# Autodesk Inventor assembly: Baugruppe1
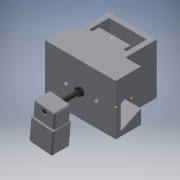
[picture p0: Inventor's stored thumbnail of the model, 180x180]
Saved by Autodesk Inventor 2017 (Build 210142000, 142)
## iProperties
Part Number: Baugruppe1
Material: Generisch
Document SubType Name: Assembly
Designer: Skenderbeg
Author: Skenderbeg
## Documents named in this file (7)
- C:\Users\Skenderbeg\Desktop\Seminar Abschluss\LaserHalterung\Baugruppe1.iam
- C:\Users\Skenderbeg\Desktop\Seminar 2018\21052018 Stick\Freiburg seminar\Schienenaufsatz mitKeil.ipt
- C:\Users\Skenderbeg\Desktop\Seminar 2018\21052018 Stick\Freiburg seminar\Schwalbenschwanz Gegenstück für Cam.ipt
- C:\Users\Skenderbeg\Desktop\Seminar 2018\21052018 Stick\Halterung Laser neu Teil2.ipt
- C:\Users\Skenderbeg\Desktop\Seminar 2018\21052018 Stick\Halterung Neu.ipt
- C:\Users\Skenderbeg\Documents\Inventor\Content Center Files\R2017\de-DE\ISO 7046-1 Z(1)\ISO 7046-1 - M4 x 40 - 4.8 - Z - ISO.ipt
- C:\Users\Skenderbeg\Documents\Inventor\Content Center Files\R2017\de-DE\ISO 4036(2)\ISO 4036 - M4(2).ipt
## Components (6 placed, 6 different names)
1. Schienenaufsatz mitKeil:1 — Verschiebbar:1
2. Schwalbenschwanz Gegenstück für Cam:1 — Verschiebbar:1, Einfügen:1, Einfügen:3
3. Halterung Laser neu Teil2:1 — Starr:1
4. Halterung Neu:1 — Starr:1, Einfügen:2
5. ISO 7046-1 Z M4 x 40 - 4.8 - Z:1 — Einfügen:1, Einfügen:2
6. ISO 4036 M4:1 — Einfügen:3
## Relationships (5: Insert 3, TranslationJoint 1, WeldJoint 1)
- Verschiebbar:1 [TranslationJoint]: Schienenaufsatz mitKeil:1 ↔ Schwalbenschwanz Gegenstück für Cam:1
- Starr:1 [WeldJoint]: Halterung Laser neu Teil2:1 ↔ Halterung Neu:1
- Einfügen:1 [Insert]: Schwalbenschwanz Gegenstück für Cam:1 ↔ ISO 7046-1 Z M4 x 40 - 4.8 - Z:1
- Einfügen:2 [Insert]: Halterung Neu:1 ↔ ISO 7046-1 Z M4 x 40 - 4.8 - Z:1
- Einfügen:3 [Insert]: Schwalbenschwanz Gegenstück für Cam:1 ↔ ISO 4036 M4:1
